# Autodesk Inventor assembly: arm
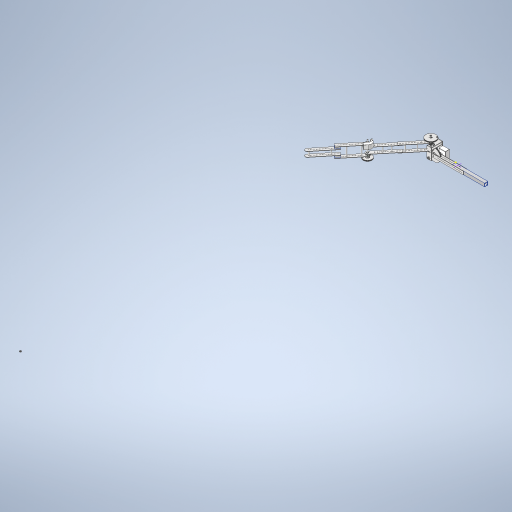
[picture p0: Inventor's stored thumbnail of the model, 512x512]
Saved by Autodesk Inventor 2024 (Build 280153000, 153)
## iProperties
Created: 2025-08-05
Part Number: arm
Document SubType Name: Assembly
Designer: HosodaLab2
Author: HosodaLab2
## Documents named in this file (46)
- C:\Users\HosodaLab2\OneDrive - Kyoto University\ドキュメント\Inventor\arm\arm.iam
- C:\Users\HosodaLab2\OneDrive - Kyoto University\ドキュメント\Inventor\arm\arm_jig.ipt
- C:\Users\HosodaLab2\OneDrive - Kyoto University\ドキュメント\Inventor\arm\elbow_stopper.ipt
- C:\Users\HosodaLab2\OneDrive - Kyoto University\ドキュメント\Inventor\arm\shoulder2_upper_plate.ipt
- C:\Users\HosodaLab2\OneDrive - Kyoto University\ドキュメント\Inventor\arm\base.ipt
- C:\Users\HosodaLab2\OneDrive - Kyoto University\ドキュメント\Inventor\arm\elbow_lower_plate.ipt
- C:\Users\HosodaLab2\OneDrive - Kyoto University\ドキュメント\Inventor\arm\elbow_upper_plate.ipt
- C:\Users\HosodaLab2\OneDrive - Kyoto University\ドキュメント\Inventor\arm\shoulder_stopper.ipt
- C:\Users\HosodaLab2\OneDrive - Kyoto University\ドキュメント\Inventor\arm\CUI_AMT102-1024-I8000-S.iam
- C:\Users\HosodaLab2\OneDrive - Kyoto University\ドキュメント\Inventor\arm\STHRANG8-MB.iam
- C:\Users\HosodaLab2\OneDrive - Kyoto University\ドキュメント\Inventor\arm\F686ZZ.ipt
- C:\Users\HosodaLab2\OneDrive - Kyoto University\ドキュメント\Inventor\arm\shoulder1_shaft.ipt
- C:\Users\HosodaLab2\OneDrive - Kyoto University\ドキュメント\Inventor\arm\shoulder2_shaft.ipt
- C:\Users\HosodaLab2\OneDrive - Kyoto University\ドキュメント\Inventor\arm\elbow_shaft.ipt
- C:\Users\HosodaLab2\OneDrive - Kyoto University\ドキュメント\Inventor\arm\pully_elbow.ipt
- C:\Users\HosodaLab2\OneDrive - Kyoto University\ドキュメント\Inventor\arm\pully_shoulder1.ipt
- C:\Users\HosodaLab2\OneDrive - Kyoto University\ドキュメント\Inventor\arm\shoulder1_upper_plate.ipt
- C:\Users\HosodaLab2\OneDrive - Kyoto University\ドキュメント\Inventor\arm\shoulder1_shaftholder_spacer_bottom.ipt
- C:\Users\HosodaLab2\OneDrive - Kyoto University\ドキュメント\Inventor\arm\shoulder1_shaftholder_spacer_upper.ipt
- C:\Users\HosodaLab2\OneDrive - Kyoto University\ドキュメント\Inventor\arm\shoulder1_upper_enocder_spacer.ipt
- C:\Users\HosodaLab2\OneDrive - Kyoto University\ドキュメント\Inventor\arm\shoulder1_under_lower_plate_spacer.ipt
- C:\Users\HosodaLab2\OneDrive - Kyoto University\ドキュメント\Inventor\arm\shoulder1_lower_cover.ipt
- C:\Users\HosodaLab2\OneDrive - Kyoto University\ドキュメント\Inventor\arm\shoulder1_upper_cover.ipt
- C:\Users\HosodaLab2\OneDrive - Kyoto University\ドキュメント\Inventor\arm\shoulder1_verticval_left_cover.ipt
- C:\Users\HosodaLab2\OneDrive - Kyoto University\ドキュメント\Inventor\arm\shoulder1_verticval_right_cover.ipt
- C:\Users\HosodaLab2\OneDrive - Kyoto University\ドキュメント\Inventor\arm\STHRANG10-MB_ss.ipt
- C:\Users\HosodaLab2\OneDrive - Kyoto University\ドキュメント\Inventor\arm\shoulder1_lower_plate.ipt
- C:\Users\HosodaLab2\OneDrive - Kyoto University\ドキュメント\Inventor\arm\F688ZZ.iam
- C:\Users\HosodaLab2\OneDrive - Kyoto University\ドキュメント\Inventor\arm\SCST6-8.iam
- C:\Users\HosodaLab2\OneDrive - Kyoto University\ドキュメント\Inventor\arm\shoulder2_upper_plate_spacer.ipt
- C:\Users\HosodaLab2\OneDrive - Kyoto University\ドキュメント\Inventor\arm\shoulder1_encorder_spacer.ipt
- C:\Users\HosodaLab2\OneDrive - Kyoto University\ドキュメント\Inventor\arm\shoulder2_encorder_spacer.ipt
- C:\Users\HosodaLab2\OneDrive - Kyoto University\ドキュメント\Inventor\arm\shoulder2_pully_spacer.ipt
- C:\Users\HosodaLab2\OneDrive - Kyoto University\ドキュメント\Inventor\arm\pully_shoulder2.ipt
- pully_shoulder_2_80.ipt
- C:\Users\HosodaLab2\OneDrive - Kyoto University\ドキュメント\Inventor\arm\shoulder2_upperplate_left_spacer.ipt
- C:\Users\HosodaLab2\OneDrive - Kyoto University\ドキュメント\Inventor\arm\shoulder2_upperplate_right_spacer.ipt
- C:\Users\HosodaLab2\OneDrive - Kyoto University\ドキュメント\Inventor\arm\shoulder2_lower_left_plate.ipt
- C:\Users\HosodaLab2\OneDrive - Kyoto University\ドキュメント\Inventor\arm\shoulder2_lower_right_plate.ipt
- C:\Users\HosodaLab2\OneDrive - Kyoto University\ドキュメント\Inventor\arm\elbow_encorder_spacer.ipt
- C:\Users\HosodaLab2\OneDrive - Kyoto University\ドキュメント\Inventor\arm\elbow_upperplate_left_spacer.ipt
- C:\Users\HosodaLab2\OneDrive - Kyoto University\ドキュメント\Inventor\arm\elbow_upperplate_right_spacer.ipt
- C:\Users\HosodaLab2\OneDrive - Kyoto University\ドキュメント\Inventor\arm\elbow_pully_spacer.ipt
- C:\Users\HosodaLab2\OneDrive - Kyoto University\ドキュメント\Inventor\arm\shoulder2_lower_plate_spacer.ipt
- C:\Users\HosodaLab2\OneDrive - Kyoto University\ドキュメント\Inventor\arm\elbow_lower_plate_spacer.ipt
- C:\Users\HosodaLab2\OneDrive - Kyoto University\ドキュメント\Inventor\arm\elbow_upper_plate_spacer.ipt
## Components (64 placed, 44 different names)
1. arm_jig:1 — 回転:140, 回転:141, 回転:142, 回転:143
2. base:1 — 回転:33, 回転:34, 回転:73, 回転:74
3. elbow_lower_plate:1 — 回転:142, 回転:143, リジッド:2, 回転:167
4. elbow_stopper:1 — 回転:168, 回転:169
5. shoulder1_encorder_spacer:1 — 回転:62, 回転:63
6. shoulder_stopper:1 — 回転:58, 回転:59
7. shoulder1_plate:1 — 回転:33, 回転:34, 角度:3, 回転:58, 回転:59, 回転:62, 回転:63, 回転:89, 角度:5
8. elbow_upper_plate:2 — 回転:140, 回転:141, 回転:144, 回転:148, 回転:149, 回転:153
9. shoulder2_lower_left_plate:1 — 回転:132, 回転:133, 角度:9, 回転:152, 回転:178, 回転:179
10. shoulder2_upper_plate:2 — 円柱状:2, メイト:1, 回転:127, 回転:128, メイト:2, 回転:173, 回転:175, 回転:178, 回転:179
11. shoulder2_lower_right_plate:1 — 回転:106, 回転:151, 回転:168, 回転:169, 回転:176, 回転:177
12. shoulder2_upper_plate:3 — 円柱状:5, 回転:122, 回転:130, 回転:172, 回転:174, 回転:176, 回転:177, 角度:10
13. arm_jig:2
14. elbow_lower_plate:3 — 回転:155, 回転:156
15. elbow_upper_plate:3 — 回転:154, 回転:161, 回転:162, 回転:163, 回転:166, リジッド:1
16. CUI_AMT102-1024-I8000-S:1 [sub-assembly] — 回転:111, 角度:8
17. CUI_AMT102-1024-I8000-S:3 [sub-assembly] — 角度:3, 回転:87, 回転:92
18. F686ZZ:1
19. shoulder1_shaft:1 — 回転:91
20. shoulder2_shaft:1 — 回転:131, 回転:135
21. pully_elbow:1 — 回転:164, 回転:165
22. pully_shoulder1:3 — 回転:157, 回転:158
23. shoulder1_shaftholder_spacer_bottom:1 — 回転:79, 回転:121
24. shoulder1_shaftholder_spacer_upper:1 — 回転:83
25. shoulder1_upper_enocder_spacer:1 — 回転:87, 回転:95, 回転:96
26. shoulder1_under_lower_plate_spacer:1 — 回転:93, 回転:109
27. shoulder1_upper_cover:1 — 回転:60, 回転:61, 回転:66, 角度:5, 回転:95, 回転:96, 回転:98, 回転:99, 回転:113, 回転:114
28. shoulder1_verticval_right_cover:1 — 回転:60, 回転:61, 回転:102, 回転:103, 回転:110, 回転:114, 角度:10
29. shoulder1_verticval_left_cover:1 — 回転:66, 回転:112, 回転:113
30. shoulder2_encorder_spacer:1 — 回転:102, 回転:103
31. STHRANG10-MB_ss:1 — 回転:79, 回転:83, 回転:157, 回転:158
32. STHRANG8-MB:2 [sub-assembly] — 回転:123, 回転:124, 円柱状:8, 回転:159
33. shoulder1_lower_plate:1 — 回転:73, 回転:74, 回転:88, 角度:7
34. F688ZZ:1 [sub-assembly] — 回転:88, 回転:93, 回転:121
35. F688ZZ:2 [sub-assembly] — 回転:89, 回転:91, 回転:92
36. SCST6-8:1 [sub-assembly] — 回転:98, 回転:99
37. SCST6-8:2 [sub-assembly]
38. shoulder2_upper_plate_spacer:1 — 回転:172, 回転:173
39. F688ZZ:3 [sub-assembly] — 回転:106, 回転:135, 回転:137
40. F688ZZ:4 [sub-assembly] — 回転:131, 回転:134
41. shoulder1_lower_cover:2 — 角度:7, 回転:109, メイト:1, 角度:8
42. F688ZZ:5 [sub-assembly] — 回転:110, 回転:111
43. F688ZZ:6 [sub-assembly] — 回転:112, 円柱状:6, 回転:129
44. shoulder1_shaftholder_spacer_bottom:2
45. shoulder2_pully_spacer:1 — 円柱状:4, 円柱状:7, 回転:122, 回転:123, 回転:124
46. pully_shoulder_2_80:1 — 円柱状:8, 回転:159
47. STHRANG8-MB:3 [sub-assembly] — 回転:127, 回転:128
48. shoulder2_upperplate_left_spacer:1 — 回転:129
49. shoulder2_upperplate_right_spacer:1 — 回転:130
50. CUI_AMT102-1024-I8000-S:4 [sub-assembly] — 回転:134, 角度:9, 回転:136
51. elbow_encorder_spacer:1 — 回転:132, 回転:133
52. elbow_upperplate_right_spacer:1 — 回転:137, 回転:144
53. elbow_upperplate_left_spacer:2 — 回転:136, 回転:162
54. elbow_pully_spacer:1 — 回転:146, 回転:147, 回転:161, 回転:163
55. STHRANG8-MB:4 [sub-assembly] — 回転:146, 回転:147, 回転:164, 回転:165
56. STHRANG8-MB:5 [sub-assembly] — 回転:148, 回転:149
57. shoulder2_upper_plate_spacer:2 — 回転:174, 回転:175
58. shoulder2_lower_plate_spacer:1 — 回転:151
59. shoulder2_lower_plate_spacer:2 — 回転:152
60. elbow_lower_plate_spacer:1 — 回転:155, リジッド:2
61. elbow_upper_plate_spacer:1 — 回転:153, 回転:166
62. elbow_upper_plate_spacer:2 — 回転:154, リジッド:1
63. elbow_lower_plate_spacer:2 — 回転:156, 回転:167
64. elbow_shaft:1 — 円柱状:2, 円柱状:4, 円柱状:5, 円柱状:6, 円柱状:7, メイト:2
## Relationships (102: RevoluteJoint 86, Angle 6, CylindricalJoint 6, Mate 2, WeldJoint 2)
- [RevoluteJoint]: arm_jig:2 ↔ elbow_upper_plate:3
- [RevoluteJoint]: arm_jig:2 ↔ elbow_upper_plate:3
- [RevoluteJoint]: arm_jig:2 ↔ elbow_lower_plate:3
- [RevoluteJoint]: arm_jig:2 ↔ elbow_lower_plate:3
- 回転:33 [RevoluteJoint]: base:1 ↔ shoulder1_plate:1
- 回転:34 [RevoluteJoint]: base:1 ↔ shoulder1_plate:1
- 角度:3 [Angle] (180 deg): shoulder1_plate:1 ↔ CUI_AMT102-1024-I8000-S:3
- 回転:58 [RevoluteJoint]: shoulder_stopper:1 ↔ shoulder1_plate:1
- 回転:59 [RevoluteJoint]: shoulder_stopper:1 ↔ shoulder1_plate:1
- 回転:60 [RevoluteJoint]: shoulder1_upper_cover:1 ↔ shoulder1_verticval_right_cover:1
- 回転:61 [RevoluteJoint]: shoulder1_upper_cover:1 ↔ shoulder1_verticval_right_cover:1
- 回転:62 [RevoluteJoint]: shoulder1_encorder_spacer:1 ↔ shoulder1_plate:1
- 回転:63 [RevoluteJoint]: shoulder1_encorder_spacer:1 ↔ shoulder1_plate:1
- 回転:66 [RevoluteJoint]: shoulder1_upper_cover:1 ↔ shoulder1_verticval_left_cover:1
- 回転:73 [RevoluteJoint]: base:1 ↔ shoulder1_lower_plate:1
- 回転:74 [RevoluteJoint]: base:1 ↔ shoulder1_lower_plate:1
- 回転:79 [RevoluteJoint]: shoulder1_shaftholder_spacer_bottom:1 ↔ STHRANG10-MB_ss:1
- 回転:83 [RevoluteJoint]: shoulder1_shaftholder_spacer_upper:1 ↔ STHRANG10-MB_ss:1
- 回転:87 [RevoluteJoint]: CUI_AMT102-1024-I8000-S:3 ↔ shoulder1_upper_enocder_spacer:1
- 回転:88 [RevoluteJoint]: shoulder1_lower_plate:1 ↔ F688ZZ:1
- 回転:89 [RevoluteJoint]: shoulder1_plate:1 ↔ F688ZZ:2
- 回転:91 [RevoluteJoint]: shoulder1_shaft:1 ↔ F688ZZ:2
- 角度:5 [Angle] (0 deg): shoulder1_plate:1 ↔ shoulder1_upper_cover:1
- 回転:92 [RevoluteJoint]: CUI_AMT102-1024-I8000-S:3 ↔ F688ZZ:2
- 回転:93 [RevoluteJoint]: shoulder1_under_lower_plate_spacer:1 ↔ F688ZZ:1
- 回転:95 [RevoluteJoint]: shoulder1_upper_enocder_spacer:1 ↔ shoulder1_upper_cover:1
- 回転:96 [RevoluteJoint]: shoulder1_upper_enocder_spacer:1 ↔ shoulder1_upper_cover:1
- 回転:98 [RevoluteJoint]: shoulder1_upper_cover:1 ↔ SCST6-8:1
- 回転:99 [RevoluteJoint]: shoulder1_upper_cover:1 ↔ SCST6-8:1
- 回転:102 [RevoluteJoint]: shoulder1_verticval_right_cover:1 ↔ shoulder2_encorder_spacer:1
- 回転:103 [RevoluteJoint]: shoulder1_verticval_right_cover:1 ↔ shoulder2_encorder_spacer:1
- 回転:106 [RevoluteJoint]: shoulder2_lower_right_plate:1 ↔ F688ZZ:3
- 角度:7 [Angle] (180 deg): shoulder1_lower_plate:1 ↔ shoulder1_lower_cover:2
- 回転:109 [RevoluteJoint]: shoulder1_under_lower_plate_spacer:1 ↔ shoulder1_lower_cover:2
- 回転:110 [RevoluteJoint]: shoulder1_verticval_right_cover:1 ↔ F688ZZ:5
- 回転:111 [RevoluteJoint]: CUI_AMT102-1024-I8000-S:1 ↔ F688ZZ:5
- 回転:112 [RevoluteJoint]: shoulder1_verticval_left_cover:1 ↔ F688ZZ:6
- 回転:113 [RevoluteJoint]: shoulder1_upper_cover:1 ↔ shoulder1_verticval_left_cover:1
- 回転:114 [RevoluteJoint]: shoulder1_upper_cover:1 ↔ shoulder1_verticval_right_cover:1
- 円柱状:2 [CylindricalJoint]: shoulder2_upper_plate:2 ↔ elbow_shaft:1
- メイト:1 [Mate] (2.5 mm): shoulder2_upper_plate:2 ↔ shoulder1_lower_cover:2
- 回転:121 [RevoluteJoint]: shoulder1_shaftholder_spacer_bottom:1 ↔ F688ZZ:1
- 角度:8 [Angle] (0 deg): CUI_AMT102-1024-I8000-S:1 ↔ shoulder1_lower_cover:2
- 円柱状:4 [CylindricalJoint]: shoulder2_pully_spacer:1 ↔ elbow_shaft:1
- 円柱状:5 [CylindricalJoint]: shoulder2_upper_plate:3 ↔ elbow_shaft:1
- 円柱状:6 [CylindricalJoint]: F688ZZ:6 ↔ elbow_shaft:1
- 円柱状:7 [CylindricalJoint]: shoulder2_pully_spacer:1 ↔ elbow_shaft:1
- 回転:122 [RevoluteJoint]: shoulder2_upper_plate:3 ↔ shoulder2_pully_spacer:1
- 回転:123 [RevoluteJoint]: STHRANG8-MB:2 ↔ shoulder2_pully_spacer:1
- 回転:124 [RevoluteJoint]: STHRANG8-MB:2 ↔ shoulder2_pully_spacer:1
- 回転:127 [RevoluteJoint]: shoulder2_upper_plate:2 ↔ STHRANG8-MB:3
- 回転:128 [RevoluteJoint]: shoulder2_upper_plate:2 ↔ STHRANG8-MB:3
- メイト:2 [Mate] (20 mm): shoulder2_upper_plate:2 ↔ elbow_shaft:1
- 回転:129 [RevoluteJoint]: F688ZZ:6 ↔ shoulder2_upperplate_left_spacer:1
- 回転:130 [RevoluteJoint]: shoulder2_upper_plate:3 ↔ shoulder2_upperplate_right_spacer:1
- 回転:131 [RevoluteJoint]: shoulder2_shaft:1 ↔ F688ZZ:4
- 回転:132 [RevoluteJoint]: shoulder2_lower_left_plate:1 ↔ elbow_encorder_spacer:1
- 回転:133 [RevoluteJoint]: shoulder2_lower_left_plate:1 ↔ elbow_encorder_spacer:1
- 回転:134 [RevoluteJoint]: F688ZZ:4 ↔ CUI_AMT102-1024-I8000-S:4
- 回転:135 [RevoluteJoint]: shoulder2_shaft:1 ↔ F688ZZ:3
- 角度:9 [Angle] (0 deg): shoulder2_lower_left_plate:1 ↔ CUI_AMT102-1024-I8000-S:4
- 回転:136 [RevoluteJoint]: CUI_AMT102-1024-I8000-S:4 ↔ elbow_upperplate_left_spacer:2
- 回転:137 [RevoluteJoint]: F688ZZ:3 ↔ elbow_upperplate_right_spacer:1
- 回転:140 [RevoluteJoint]: arm_jig:1 ↔ elbow_upper_plate:2
- 回転:141 [RevoluteJoint]: arm_jig:1 ↔ elbow_upper_plate:2
- 回転:142 [RevoluteJoint]: arm_jig:1 ↔ elbow_lower_plate:1
- 回転:143 [RevoluteJoint]: arm_jig:1 ↔ elbow_lower_plate:1
- 回転:144 [RevoluteJoint]: elbow_upper_plate:2 ↔ elbow_upperplate_right_spacer:1
- 回転:146 [RevoluteJoint]: elbow_pully_spacer:1 ↔ STHRANG8-MB:4
- 回転:147 [RevoluteJoint]: elbow_pully_spacer:1 ↔ STHRANG8-MB:4
- 回転:148 [RevoluteJoint]: elbow_upper_plate:2 ↔ STHRANG8-MB:5
- 回転:149 [RevoluteJoint]: elbow_upper_plate:2 ↔ STHRANG8-MB:5
- 回転:151 [RevoluteJoint]: shoulder2_lower_right_plate:1 ↔ shoulder2_lower_plate_spacer:1
- 回転:152 [RevoluteJoint]: shoulder2_lower_left_plate:1 ↔ shoulder2_lower_plate_spacer:2
- 回転:153 [RevoluteJoint]: elbow_upper_plate:2 ↔ elbow_upper_plate_spacer:1
- 回転:154 [RevoluteJoint]: elbow_upper_plate:3 ↔ elbow_upper_plate_spacer:2
- 回転:155 [RevoluteJoint]: elbow_lower_plate:3 ↔ elbow_lower_plate_spacer:1
- 回転:156 [RevoluteJoint]: elbow_lower_plate:3 ↔ elbow_lower_plate_spacer:2
- 回転:157 [RevoluteJoint]: pully_shoulder1:3 ↔ STHRANG10-MB_ss:1
- 回転:158 [RevoluteJoint]: pully_shoulder1:3 ↔ STHRANG10-MB_ss:1
- 円柱状:8 [CylindricalJoint]: STHRANG8-MB:2 ↔ pully_shoulder_2_80:1
- 回転:159 [RevoluteJoint]: STHRANG8-MB:2 ↔ pully_shoulder_2_80:1
- 回転:161 [RevoluteJoint]: elbow_upper_plate:3 ↔ elbow_pully_spacer:1
- 回転:162 [RevoluteJoint]: elbow_upper_plate:3 ↔ elbow_upperplate_left_spacer:2
- 回転:163 [RevoluteJoint]: elbow_upper_plate:3 ↔ elbow_pully_spacer:1
- 回転:164 [RevoluteJoint]: pully_elbow:1 ↔ STHRANG8-MB:4
- 回転:165 [RevoluteJoint]: pully_elbow:1 ↔ STHRANG8-MB:4
- 回転:166 [RevoluteJoint]: elbow_upper_plate:3 ↔ elbow_upper_plate_spacer:1
- リジッド:1 [WeldJoint]: elbow_upper_plate:3 ↔ elbow_upper_plate_spacer:2
- リジッド:2 [WeldJoint]: elbow_lower_plate:1 ↔ elbow_lower_plate_spacer:1
- 回転:167 [RevoluteJoint]: elbow_lower_plate:1 ↔ elbow_lower_plate_spacer:2
- 回転:168 [RevoluteJoint]: elbow_stopper:1 ↔ shoulder2_lower_right_plate:1
- 回転:169 [RevoluteJoint]: elbow_stopper:1 ↔ shoulder2_lower_right_plate:1
- 回転:172 [RevoluteJoint]: shoulder2_upper_plate:3 ↔ shoulder2_upper_plate_spacer:1
- 回転:173 [RevoluteJoint]: shoulder2_upper_plate:2 ↔ shoulder2_upper_plate_spacer:1
- 回転:174 [RevoluteJoint]: shoulder2_upper_plate:3 ↔ shoulder2_upper_plate_spacer:2
- 回転:175 [RevoluteJoint]: shoulder2_upper_plate:2 ↔ shoulder2_upper_plate_spacer:2
- 回転:176 [RevoluteJoint]: shoulder2_lower_right_plate:1 ↔ shoulder2_upper_plate:3
- 回転:177 [RevoluteJoint]: shoulder2_lower_right_plate:1 ↔ shoulder2_upper_plate:3
- 回転:178 [RevoluteJoint]: shoulder2_lower_left_plate:1 ↔ shoulder2_upper_plate:2
- 回転:179 [RevoluteJoint]: shoulder2_lower_left_plate:1 ↔ shoulder2_upper_plate:2
- 角度:10 [Angle] (180 deg): shoulder2_upper_plate:3 ↔ shoulder1_verticval_right_cover:1
## Named parameters: d38_d30 = 0 mm, d39_d31 = 90 deg, d40_d32 = 0 mm, d41_d33 = 90 deg, d42_d34 = 0 mm, d43_d35 = 180 deg, d44_d36 = 0 mm, d45_d37 = -90 deg
